# Autodesk Inventor assembly: Top_Rail_Full
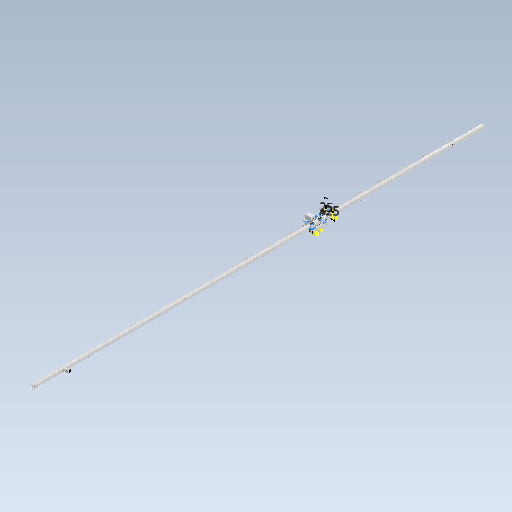
[picture p0: Inventor's stored thumbnail of the model, 512x512]
Saved by Autodesk Inventor 2021 (Build 250183000, 183)
## iProperties
Created: 2022-01-15
Part Number: Top_Rail_Full
Document SubType Name: Assembly
Designer: Jorian Brusind
Description: Top rail assembly for y axis
Author: Jorian Brusind
Revision Number: 2.0
## Documents named in this file (11)
- C:\Users\Jorian Brusind\Documents\GitHub\HyperRail\Inventor Files\Top_Rail_Full.iam
- C:\Users\Jorian Brusind\Documents\GitHub\HyperRail\Inventor Files\Top_Rail_Section.iam
- C:\Users\Jorian Brusind\Documents\GitHub\HyperRail\Inventor Files\MagnetActuatorHolder.ipt
- C:\Users\Jorian Brusind\Documents\GitHub\HyperRail\Inventor Files\MagnetHolder.ipt
- C:\Users\Jorian Brusind\Documents\GitHub\HyperRail\Inventor Files\59145_Sensor.ipt
- C:\Users\Jorian Brusind\Documents\GitHub\HyperRail\Inventor Files\McMaster Files\Belts\7959K23_1 2 Width MXL Series No. Ll050mxl Timing Belt_20ft.ipt
- C:\Users\Jorian Brusind\Documents\GitHub\HyperRail\Inventor Files\CableChain_Holder.ipt
- C:\Users\Jorian Brusind\Documents\GitHub\HyperRail\Inventor Files\YAxis_Carriage.iam
- C:\Users\Jorian Brusind\Documents\GitHub\HyperRail\Inventor Files\CableChain_Clamp.iam
- C:\Users\Jorian Brusind\Documents\GitHub\HyperRail\Inventor Files\17mmBeltGuide.ipt
- C:\Users\Jorian Brusind\Documents\GitHub\HyperRail\Inventor Files\McMaster Files\Belts\7959K23_1 2 Width MXL Series No. Ll050mxl Timing Belt_small.ipt
## Components (22 placed, 10 different names)
1. Top_Rail_Section:1 [sub-assembly] — Mate:2, Flush:3, Flush:4, Flush:6
2. Top_Rail_Section:2 [sub-assembly] — Mate:1, Flush:1, Flush:2, Mate:2, Flush:3, Flush:4, Mate:10, Mate:12
3. Top_Rail_Section:3 [sub-assembly] — Mate:1, Flush:1, Flush:2, Mate:3, Flush:5, Mate:6, Flush:8, Mate:11, Flush:9, Flush:10, Flush:11, Mate:13, Mate:14, Flush:12, Mate:17, Mate:18, Mate:19, Flush:15
4. MagnetActuatorHolder:1 — Mate:3, Flush:5, Flush:6, Mate:8, Mate:9, Angle:2
5. MagnetHolder:1 — Mate:4, Mate:5, Angle:1, Mate:6, Flush:11, Flush:15
6. 59145_Sensor:1 — Mate:4, Mate:5, Angle:1
7. 59145_Sensor:2 — Mate:8, Mate:9, Angle:2
8. 7959K23_1 2 Width MXL Series No. Ll050mxl Timing Belt_20ft:1 — Mate:10, Flush:8, Flush:12, Flush:13, Mate:21
9. YAxis_Carriage:1 [sub-assembly] — Mate:12, Mate:13, Mate:14, Mate:16, Angle:3, Flush:14
10. CableChain_Clamp:1 [sub-assembly] — Mate:17, Mate:18, Mate:19, Mate:20
11. 17mmBeltGuide:1 — Mate:15, Mate:16, Angle:3, Mate:20
12. 7959K23_1 2 Width MXL Series No. Ll050mxl Timing Belt_small:1 — Flush:13, Mate:21, Flush:14
13. CableChain_Holder:1 — Mate:11, Flush:9, Flush:10
14. CableChain_Holder:2
15. CableChain_Holder:3
16. CableChain_Holder:4
17. CableChain_Holder:5
18. CableChain_Holder:6 — Mate:15
19. CableChain_Holder:7
20. CableChain_Holder:8
21. CableChain_Holder:9
22. CableChain_Holder:10
## Component patterns: (10 elements, first: CableChain_Holder:1)
## Relationships (37: Mate 20, Flush 14, Angle 3)
- Mate:1: Top_Rail_Section:2 ↔ Top_Rail_Section:3
- Flush:1: Top_Rail_Section:2 ↔ Top_Rail_Section:3
- Flush:2: Top_Rail_Section:2 ↔ Top_Rail_Section:3
- Mate:2: Top_Rail_Section:1 ↔ Top_Rail_Section:2
- Flush:3: Top_Rail_Section:1 ↔ Top_Rail_Section:2
- Flush:4: Top_Rail_Section:1 ↔ Top_Rail_Section:2
- Mate:3: Top_Rail_Section:3 ↔ MagnetActuatorHolder:1
- Flush:5: Top_Rail_Section:3 ↔ MagnetActuatorHolder:1
- Mate:4: MagnetHolder:1 ↔ 59145_Sensor:1
- Mate:5: MagnetHolder:1 ↔ 59145_Sensor:1
- Angle:1 (0 deg): MagnetHolder:1 ↔ 59145_Sensor:1
- Mate:6: Top_Rail_Section:3 ↔ MagnetHolder:1
- Flush:6 (400 mm): Top_Rail_Section:1 ↔ MagnetActuatorHolder:1
- Mate:8: MagnetActuatorHolder:1 ↔ 59145_Sensor:2
- Mate:9: MagnetActuatorHolder:1 ↔ 59145_Sensor:2
- Angle:2 (0 deg): MagnetActuatorHolder:1 ↔ 59145_Sensor:2
- Mate:10: Top_Rail_Section:2 ↔ 7959K23_1 2 Width MXL Series No. Ll050mxl Timing Belt_20ft:1
- Flush:8: Top_Rail_Section:3 ↔ 7959K23_1 2 Width MXL Series No. Ll050mxl Timing Belt_20ft:1
- Mate:11: Top_Rail_Section:3 ↔ CableChain_Holder:1
- Flush:9: Top_Rail_Section:3 ↔ CableChain_Holder:1
- Flush:10 (400 mm): Top_Rail_Section:3 ↔ CableChain_Holder:1
- Flush:11 (400 mm): Top_Rail_Section:3 ↔ MagnetHolder:1
- Mate:12 (12 mm): Top_Rail_Section:2 ↔ YAxis_Carriage:1
- Mate:13 (22 mm): Top_Rail_Section:3 ↔ YAxis_Carriage:1
- Mate:14 (12 mm): Top_Rail_Section:3 ↔ YAxis_Carriage:1
- Flush:12 (5 mm): Top_Rail_Section:3 ↔ 7959K23_1 2 Width MXL Series No. Ll050mxl Timing Belt_20ft:1
- Mate:15: 17mmBeltGuide:1 ↔ CableChain_Holder:6
- Mate:16: YAxis_Carriage:1 ↔ 17mmBeltGuide:1
- Angle:3 (0 deg): YAxis_Carriage:1 ↔ 17mmBeltGuide:1
- Mate:17 (12 mm): Top_Rail_Section:3 ↔ CableChain_Clamp:1
- Mate:18 (12 mm): Top_Rail_Section:3 ↔ CableChain_Clamp:1
- Mate:19 (20 mm): Top_Rail_Section:3 ↔ CableChain_Clamp:1
- Mate:20 (18 mm): CableChain_Clamp:1 ↔ 17mmBeltGuide:1
- Flush:13: 7959K23_1 2 Width MXL Series No. Ll050mxl Timing Belt_20ft:1 ↔ 7959K23_1 2 Width MXL Series No. Ll050mxl Timing Belt_small:1
- Mate:21: 7959K23_1 2 Width MXL Series No. Ll050mxl Timing Belt_20ft:1 ↔ 7959K23_1 2 Width MXL Series No. Ll050mxl Timing Belt_small:1
- Flush:14: YAxis_Carriage:1 ↔ 7959K23_1 2 Width MXL Series No. Ll050mxl Timing Belt_small:1
- Flush:15: Top_Rail_Section:3 ↔ MagnetHolder:1
